# Autodesk Inventor assembly: Y
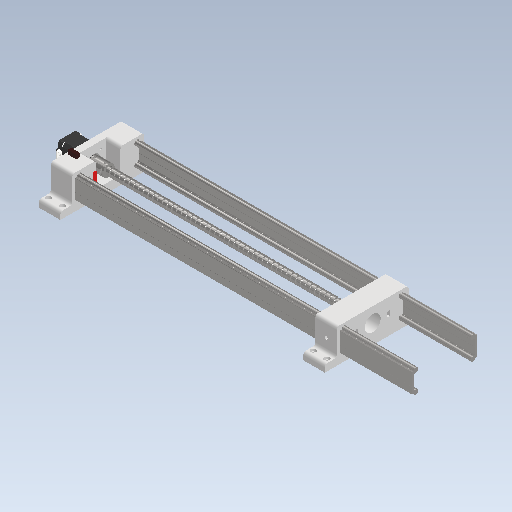
[picture p0: Inventor's stored thumbnail of the model, 512x512]
Saved by Autodesk Inventor 2020 (Build 240168000, 168)
## iProperties
Created: 2022-04-26
Part Number: Y
Document SubType Name: Assembly
Designer: mikoma
Author: mikoma
## Documents named in this file (13)
- D:\KONIECTEGOKOŁCHOZU\MGR\model\Workspaces\Obszar roboczy\assembly_v3\Y\Y.iam
- D:\KONIECTEGOKOŁCHOZU\MGR\model\Workspaces\Obszar roboczy\assembly_v3\Y\YMotorMount.ipt
- D:\KONIECTEGOKOŁCHOZU\MGR\model\Workspaces\Obszar roboczy\assembly_v3\Y\WS_10_40_Y.ipt
- D:\KONIECTEGOKOŁCHOZU\MGR\model\Workspaces\Obszar roboczy\assembly_v3\Y\YFloating.ipt
- D:\KONIECTEGOKOŁCHOZU\MGR\model\Workspaces\Obszar roboczy\content\nema17\Nema17 Stepper Motor.ipt
- D:\KONIECTEGOKOŁCHOZU\MGR\model\Workspaces\Obszar roboczy\content\manipulatorSharedParts\Cartesian1_BallScrew.ipt
- D:\KONIECTEGOKOŁCHOZU\MGR\model\Workspaces\Obszar roboczy\content\manipulatorSharedParts\Cartesian2_BallBearing_25x37x7.ipt
- D:\KONIECTEGOKOŁCHOZU\MGR\model\Workspaces\Obszar roboczy\content\manipulatorSharedParts\Cartesian1_12_12_Clutch.ipt
- D:\KONIECTEGOKOŁCHOZU\MGR\model\Workspaces\Obszar roboczy\content\manipulatorSharedParts\endCup.ipt
- D:\KONIECTEGOKOŁCHOZU\MGR\model\Workspaces\Obszar roboczy\content\manipulatorSharedParts\stopSw.ipt
- D:\KONIECTEGOKOŁCHOZU\MGR\model\Workspaces\Obszar roboczy\CC\pl-PL\ISO 4762(2)\ISO 4762 - M3 x 16ISO.ipt
- D:\KONIECTEGOKOŁCHOZU\MGR\model\Workspaces\Obszar roboczy\CC\pl-PL\DIN EN ISO 4032\DIN EN ISO 4032 - M3.ipt
- D:\KONIECTEGOKOŁCHOZU\MGR\model\Workspaces\Obszar roboczy\content\manipulatorSharedParts\Connector_female.ipt
## Components (13 placed, 12 different names)
1. YMotorMount:1 — Zestawiające:1, Równoległe:1, Zestawiające:2, Zestawiające:17, Zestawiające:18, Zestawiające:19, Kątowe:1, Zestawiające:32, Zestawiające:33, Zestawiające:34, Kątowe:2, Zestawiające:38, Zestawiające:39, Zestawiające:40, Zestawiające:41, Zestawiające:42, Zestawiające:43, Zestawiające:44, Zestawiające:45, Równoległe:6, Równoległe:7, Zestawiające:46
2. WS_10_40_Y:1 — Zestawiające:9, Zestawiające:43, Zestawiające:44, Równoległe:7
3. WS_10_40_Y:2 — Zestawiające:10, Zestawiające:42, Zestawiające:45, Równoległe:6
4. YFloating:1 — Zestawiające:9, Zestawiające:10, Zestawiające:24, Zestawiające:25
5. Nema17 Stepper Motor:1 — Zestawiające:17, Zestawiające:18, Kątowe:1
6. Cartesian1_BallScrew:1 — Zestawiające:20, Zestawiające:21
7. Cartesian2_BallBearing_25x37x7:1 — Zestawiające:24, Zestawiające:25, Zestawiające:30, Zestawiające:31
8. Cartesian1_12_12_Clutch:1 — Zestawiające:19, Zestawiające:20, Zestawiające:21, Zestawiające:46
9. endCup:1 — Zestawiające:30, Zestawiające:31
10. stopSw:1 — Zestawiające:32, Zestawiające:33, Zestawiające:34, Zestawiające:35, Zestawiające:36
11. ISO 4762 M3 x 16:1 — Zestawiające:35, Zestawiające:36, Zestawiające:37
12. DIN EN ISO 4032 M3:1 — Zestawiające:37, Kątowe:2, Zestawiające:38
13. Connector_female:1 — Zestawiające:39, Zestawiające:40, Zestawiające:41
## Relationships (33: Mate 28, Flush 3, Angle 2)
- Zestawiające:1 [Mate]: YMotorMount:1
- Równoległe:1 [Flush]: YMotorMount:1
- Zestawiające:2 [Mate]: YMotorMount:1
- Zestawiające:9 [Mate]: WS_10_40_Y:1 ↔ YFloating:1
- Zestawiające:10 [Mate]: WS_10_40_Y:2 ↔ YFloating:1
- Zestawiające:17 [Mate]: YMotorMount:1 ↔ Nema17 Stepper Motor:1
- Zestawiające:18 [Mate]: YMotorMount:1 ↔ Nema17 Stepper Motor:1
- Zestawiające:19 [Mate]: YMotorMount:1 ↔ Cartesian1_12_12_Clutch:1
- Zestawiające:20 [Mate]: Cartesian1_BallScrew:1 ↔ Cartesian1_12_12_Clutch:1
- Zestawiające:21 [Mate]: Cartesian1_BallScrew:1 ↔ Cartesian1_12_12_Clutch:1
- Zestawiające:24 [Mate]: YFloating:1 ↔ Cartesian2_BallBearing_25x37x7:1
- Zestawiające:25 [Mate]: YFloating:1 ↔ Cartesian2_BallBearing_25x37x7:1
- Zestawiające:30 [Mate]: Cartesian2_BallBearing_25x37x7:1 ↔ endCup:1
- Zestawiające:31 [Mate]: Cartesian2_BallBearing_25x37x7:1 ↔ endCup:1
- Kątowe:1 [Angle] (0 deg): YMotorMount:1 ↔ Nema17 Stepper Motor:1
- Zestawiające:32 [Mate]: YMotorMount:1 ↔ stopSw:1
- Zestawiające:33 [Mate]: YMotorMount:1 ↔ stopSw:1
- Zestawiające:34 [Mate]: YMotorMount:1 ↔ stopSw:1
- Zestawiające:35 [Mate]: stopSw:1 ↔ ISO 4762 M3 x 16:1
- Zestawiające:36 [Mate]: stopSw:1 ↔ ISO 4762 M3 x 16:1
- Zestawiające:37 [Mate]: ISO 4762 M3 x 16:1 ↔ DIN EN ISO 4032 M3:1
- Kątowe:2 [Angle] (0 deg): YMotorMount:1 ↔ DIN EN ISO 4032 M3:1
- Zestawiające:38 [Mate]: YMotorMount:1 ↔ DIN EN ISO 4032 M3:1
- Zestawiające:39 [Mate]: YMotorMount:1 ↔ Connector_female:1
- Zestawiające:40 [Mate]: YMotorMount:1 ↔ Connector_female:1
- Zestawiające:41 [Mate]: YMotorMount:1 ↔ Connector_female:1
- Zestawiające:42 [Mate]: YMotorMount:1 ↔ WS_10_40_Y:2
- Zestawiające:43 [Mate]: YMotorMount:1 ↔ WS_10_40_Y:1
- Zestawiające:44 [Mate]: YMotorMount:1 ↔ WS_10_40_Y:1
- Zestawiające:45 [Mate]: YMotorMount:1 ↔ WS_10_40_Y:2
- Równoległe:6 [Flush]: YMotorMount:1 ↔ WS_10_40_Y:2
- Równoległe:7 [Flush]: YMotorMount:1 ↔ WS_10_40_Y:1
- Zestawiające:46 [Mate]: YMotorMount:1 ↔ Cartesian1_12_12_Clutch:1
